# Autodesk Inventor assembly: ArcadeController
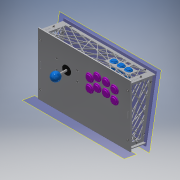
[picture p0: Inventor's stored thumbnail of the model, 180x180]
Saved by Autodesk Inventor 2019 (Build 230136000, 136)
## iProperties
Created: 2013-02-02
Part Number: ArcadeController
Document SubType Name: Assembly
Designer: xylzlyx
Author: xylzlyx
## Documents named in this file (16)
- D:\GitRepos\Pew-Pew-Stick\inventor\assemblies\ArcadeController.iam
- D:\GitRepos\Pew-Pew-Stick\inventor\parts\Panel_top.ipt
- D:\GitRepos\Pew-Pew-Stick\inventor\parts\Panel_bottom.ipt
- D:\GitRepos\Pew-Pew-Stick\inventor\parts\JLF-TP-8YT_body.ipt
- D:\GitRepos\Pew-Pew-Stick\inventor\parts\JLF-TP-8YT_ball.ipt
- D:\GitRepos\Pew-Pew-Stick\inventor\parts\JLF-TP-8YT_ring.ipt
- D:\GitRepos\Pew-Pew-Stick\inventor\parts\OBSF-30-B_button.ipt
- D:\GitRepos\Pew-Pew-Stick\inventor\parts\Panel_back.ipt
- D:\GitRepos\Pew-Pew-Stick\inventor\parts\Panel_front.ipt
- D:\GitRepos\Pew-Pew-Stick\inventor\parts\Panel_side.ipt
- D:\GitRepos\Pew-Pew-Stick\inventor\parts\OBSF-24_button.ipt
- D:\GitRepos\Pew-Pew-Stick\inventor\assemblies\ArcadeController\Design Accelerator\Bolted Connection2.iam
- D:\GitRepos\Pew-Pew-Stick\inventor\assemblies\ArcadeController\Design Accelerator\Panel Bolted Connection1.iam
- D:\GitRepos\Pew-Pew-Stick\inventor\assemblies\ArcadeController\Design Accelerator\Panel Bolted Connection2.iam
- D:\GitRepos\Pew-Pew-Stick\inventor\assemblies\ArcadeController\Design Accelerator\Front Panel Connection1.iam
- D:\GitRepos\Pew-Pew-Stick\inventor\assemblies\ArcadeController\Design Accelerator\Front Panel Connection2.iam
## Components (25 placed, 15 different names)
1. TopPanel:1 — Flush:1, Flush:2, Insert:1, Insert:2, Insert:4, Insert:5, Insert:6, Insert:7, Insert:8, Insert:9, Insert:10, Insert:11, Insert:12, Mate:6, Mate:10, Mate:14, Mate:15, Mate:16, Mate:17
2. BottomPanel:1 — Flush:1, Flush:2, Mate:3, Flush:3, Flush:4, Flush:5, Flush:6, Flush:8, Flush:9, Mate:4, Mate:5, Flush:10, Flush:12, Flush:13, Mate:8, Flush:14, Mate:13, Mate:22, Mate:23
3. JLF-TP-8YT_body:1 — Insert:1, Insert:2, Insert:3, Mate:3
4. JoystickBall:1 — Insert:3
5. JoystickCover:1 — Insert:4
6. OBSF-30-B_button:1 — Insert:5
7. OBSF-30-B_button:2 — Insert:6
8. OBSF-30-B_button:3 — Insert:7
9. OBSF-30-B_button:4 — Insert:8
10. OBSF-30-B_button:5 — Insert:9
11. OBSF-30-B_button:6 — Insert:10
12. OBSF-30-B_button:7 — Insert:11
13. OBSF-30-B_button:8 — Insert:12
14. Panel_back:1 — Flush:3, Flush:4, Mate:5, Flush:10, Mate:11, Mate:12, Insert:45, Insert:46, Insert:47, Mate:18, Mate:19
15. Panel_front:1 — Flush:5, Flush:6, Flush:12, Mate:9, Flush:14, Mate:13, Mate:20, Mate:21
16. Panel_side:1 — Flush:8, Flush:9, Mate:4, Mate:6, Mate:12
17. Panel_side:2 — Flush:13, Mate:8, Mate:9, Mate:10, Mate:11
18. OBSF-24_button:1 — Insert:45
19. OBSF-24_button:2 — Insert:46
20. OBSF-24_button:3 — Insert:47
21. Joystick Connection:1 [sub-assembly] — Mate:14, Mate:15
22. Top Panel Connection:1 [sub-assembly] — Mate:16, Mate:17
23. Back Panel Connection:1 [sub-assembly] — Mate:18, Mate:19
24. Front Panel Connection:1 [sub-assembly] — Mate:20, Mate:21
25. Bottom Panel Connection:1 [sub-assembly] — Mate:22, Mate:23
## Relationships (47: Mate 20, Insert 15, Flush 12)
- Flush:1: TopPanel:1 ↔ BottomPanel:1
- Flush:2: TopPanel:1 ↔ BottomPanel:1
- Insert:1: TopPanel:1 ↔ JLF-TP-8YT_body:1
- Insert:2: TopPanel:1 ↔ JLF-TP-8YT_body:1
- Insert:3: JLF-TP-8YT_body:1 ↔ JoystickBall:1
- Insert:4: TopPanel:1 ↔ JoystickCover:1
- Insert:5: TopPanel:1 ↔ OBSF-30-B_button:1
- Insert:6: TopPanel:1 ↔ OBSF-30-B_button:2
- Insert:7: TopPanel:1 ↔ OBSF-30-B_button:3
- Insert:8: TopPanel:1 ↔ OBSF-30-B_button:4
- Insert:9: TopPanel:1 ↔ OBSF-30-B_button:5
- Insert:10: TopPanel:1 ↔ OBSF-30-B_button:6
- Insert:11: TopPanel:1 ↔ OBSF-30-B_button:7
- Insert:12: TopPanel:1 ↔ OBSF-30-B_button:8
- Mate:3 (44.45 mm): BottomPanel:1 ↔ JLF-TP-8YT_body:1
- Flush:3: BottomPanel:1 ↔ Panel_back:1
- Flush:4 (-12.7 mm): BottomPanel:1 ↔ Panel_back:1
- Flush:5: BottomPanel:1 ↔ Panel_front:1
- Flush:6 (-9.525 mm): BottomPanel:1 ↔ Panel_front:1
- Flush:8 (-9.525 mm): BottomPanel:1 ↔ Panel_side:1
- Flush:9 (9.525 mm): BottomPanel:1 ↔ Panel_side:1
- Mate:4: BottomPanel:1 ↔ Panel_side:1
- Mate:5: BottomPanel:1 ↔ Panel_back:1
- Flush:10: BottomPanel:1 ↔ Panel_back:1
- Mate:6: TopPanel:1 ↔ Panel_side:1
- Flush:12 (9.525 mm): BottomPanel:1 ↔ Panel_front:1
- Flush:13 (9.525 mm): BottomPanel:1 ↔ Panel_side:2
- Mate:8: BottomPanel:1 ↔ Panel_side:2
- Mate:9: Panel_front:1 ↔ Panel_side:2
- Mate:10: TopPanel:1 ↔ Panel_side:2
- Mate:11: Panel_back:1 ↔ Panel_side:2
- Mate:12: Panel_back:1 ↔ Panel_side:1
- Flush:14: BottomPanel:1 ↔ Panel_front:1
- Mate:13: BottomPanel:1 ↔ Panel_front:1
- Insert:45: Panel_back:1 ↔ OBSF-24_button:1
- Insert:46: Panel_back:1 ↔ OBSF-24_button:2
- Insert:47: Panel_back:1 ↔ OBSF-24_button:3
- Mate:14: TopPanel:1 ↔ Joystick Connection:1
- Mate:15: TopPanel:1 ↔ Joystick Connection:1
- Mate:16: TopPanel:1 ↔ Top Panel Connection:1
- Mate:17: TopPanel:1 ↔ Top Panel Connection:1
- Mate:18: Panel_back:1 ↔ Back Panel Connection:1
- Mate:19: Panel_back:1 ↔ Back Panel Connection:1
- Mate:20: Panel_front:1 ↔ Front Panel Connection:1
- Mate:21: Panel_front:1 ↔ Front Panel Connection:1
- Mate:22: BottomPanel:1 ↔ Bottom Panel Connection:1
- Mate:23: BottomPanel:1 ↔ Bottom Panel Connection:1
